# Autodesk Inventor assembly: Arm Assembly
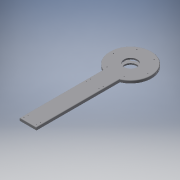
[picture p0: Inventor's stored thumbnail of the model, 180x180]
Saved by Autodesk Inventor 2016 (Build 200138000, 138)
## iProperties
Created: 2016-04-16
Part Number: Arm Assembly
Document SubType Name: Assembly
Designer: rmarkowi
Author: rmarkowi
## Documents named in this file (5)
- C:\Users\rmarkowi\Documents\GGC\V1\Arm Assembly.iam
- C:\Users\rmarkowi\Documents\GGC\V1\Arm Layer 1.ipt
- C:\Users\rmarkowi\Documents\GGC\V1\Turntable_2.ipt
- C:\Users\rmarkowi\Documents\GGC\V1\Arm Layer 2 Out.ipt
- C:\Users\rmarkowi\Documents\GGC\V1\Arm Mount.ipt
## Components (4 placed, 4 different names)
1. Arm Layer 1:1 — Mate:1, Mate:2, Mate:3, Flush:1, Mate:4, Flush:2, Mate:6
2. Turntable_2:1 — Mate:1, Mate:2, Mate:3, Mate:5, Mate:7
3. Arm Layer 2 Out:1 — Flush:1, Mate:4, Flush:2
4. Arm Mount:1 — Mate:5, Mate:6, Mate:7
## Relationships (9: Mate 7, Flush 2)
- Mate:1: Arm Layer 1:1 ↔ Turntable_2:1
- Mate:2: Arm Layer 1:1 ↔ Turntable_2:1
- Mate:3: Arm Layer 1:1 ↔ Turntable_2:1
- Flush:1: Arm Layer 1:1 ↔ Arm Layer 2 Out:1
- Mate:4: Arm Layer 1:1 ↔ Arm Layer 2 Out:1
- Flush:2: Arm Layer 1:1 ↔ Arm Layer 2 Out:1
- Mate:5 (12.7 mm): Turntable_2:1 ↔ Arm Mount:1
- Mate:6: Arm Layer 1:1 ↔ Arm Mount:1
- Mate:7: Turntable_2:1 ↔ Arm Mount:1
